# Autodesk Inventor assembly: SACMI PH1500
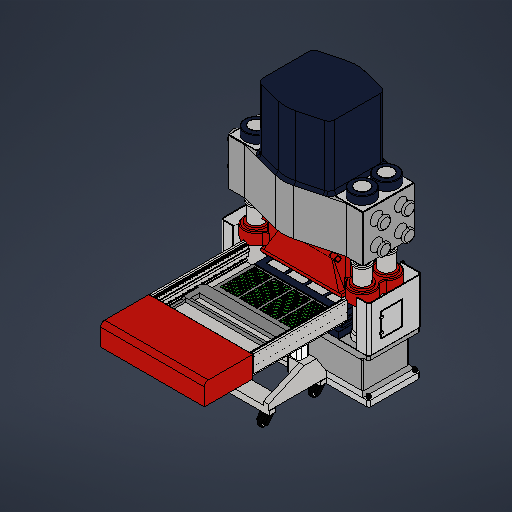
[picture p0: Inventor's stored thumbnail of the model, 512x512]
Saved by Autodesk Inventor 2025 (Build 290162000, 162)
## iProperties
Created: 2024-05-02
Part Number: SACMI PH1500
Document SubType Name: Assembly
Designer: zulet
Author: zulet
## Documents named in this file (8)
- D:\UNAL\2024-1S\APM\Digital Factory\SACMI PH1500.iam
- D:\UNAL\2024-1S\APM\Digital Factory\SACMI PH1500 30X60 DIE SET BASE.ipt
- D:\UNAL\2024-1S\APM\Digital Factory\SACMI PH1500 BASE.ipt
- D:\UNAL\2024-1S\APM\Digital Factory\SACMI PH1500 30X60 DIE SET TILES BOTTOM MOLD.ipt
- D:\UNAL\2024-1S\APM\Digital Factory\SACMI PH1500 PRESS TOP.ipt
- D:\UNAL\2024-1S\APM\Digital Factory\SACMI PH1500 30X60 DIE SET TOP.ipt
- D:\UNAL\2024-1S\APM\Digital Factory\SACMI PH1500 POWER FEED SYSTEM.ipt
- D:\UNAL\2024-1S\APM\Digital Factory\SACMI PH1500 FILLER BOX GRID-DRIVING.ipt
## Components (7 placed, 7 different names)
1. SACMI PH1500 30X60 DIE SET BASE:1 — Mate:1, Flush:1, Flush:2, Slider:1, Rigid:2
2. SACMI PH1500 BASE:1 — Mate:1, Flush:1, Flush:2, Cylindrical:1, Cylindrical:2
3. SACMI PH1500 30X60 DIE SET TILES BOTTOM MOLD:1 — Slider:1
4. SACMI PH1500 PRESS TOP:1 — Cylindrical:1, Cylindrical:2, Rigid:1
5. SACMI PH1500 30X60 DIE SET TOP:1 — Rigid:1
6. SACMI PH1500 POWER FEED SYSTEM:1 — Rigid:2, Slider:2
7. SACMI PH1500 FILLER BOX GRID-DRIVING:1 — Slider:2
## Relationships (9: Flush 2, TranslationJoint 2, CylindricalJoint 2, WeldJoint 2, Mate 1)
- Mate:1: SACMI PH1500 30X60 DIE SET BASE:1 ↔ SACMI PH1500 BASE:1
- Flush:1: SACMI PH1500 30X60 DIE SET BASE:1 ↔ SACMI PH1500 BASE:1
- Flush:2: SACMI PH1500 30X60 DIE SET BASE:1 ↔ SACMI PH1500 BASE:1
- Slider:1 [TranslationJoint]: SACMI PH1500 30X60 DIE SET BASE:1 ↔ SACMI PH1500 30X60 DIE SET TILES BOTTOM MOLD:1
- Cylindrical:1: SACMI PH1500 BASE:1 ↔ SACMI PH1500 PRESS TOP:1
- Cylindrical:2: SACMI PH1500 BASE:1 ↔ SACMI PH1500 PRESS TOP:1
- Rigid:1 [WeldJoint]: SACMI PH1500 PRESS TOP:1 ↔ SACMI PH1500 30X60 DIE SET TOP:1
- Rigid:2 [WeldJoint]: SACMI PH1500 30X60 DIE SET BASE:1 ↔ SACMI PH1500 POWER FEED SYSTEM:1
- Slider:2 [TranslationJoint]: SACMI PH1500 POWER FEED SYSTEM:1 ↔ SACMI PH1500 FILLER BOX GRID-DRIVING:1
